# Autodesk Inventor assembly: Shoulder base
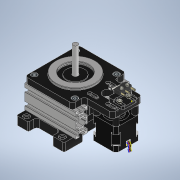
[picture p0: Inventor's stored thumbnail of the model, 180x180]
Saved by Autodesk Inventor 2022 (Build 260153000, 153)
## iProperties
Created: 2022-03-02
Part Number: Shoulder base
Document SubType Name: Assembly
Designer: JK
Author: JK
## Documents named in this file (23)
- C:\Users\JK\Documents\Inventor\ScaraNema\SCARA-3DP\Parts\Shoulder\Shoulder base.iam
- C:\Users\JK\Documents\Inventor\ScaraNema\SCARA-3DP\Parts\Shoulder\Needle roller bearing\5909K79_1 mm Thick Washer for 45 mm Shaft Diameter Needle-Roller Thrust Bearing.ipt
- C:\Users\JK\Documents\Inventor\ScaraNema\SCARA-3DP\Parts\Shoulder\Needle roller bearing\5909K19_Needle-Roller Thrust Bearing.ipt
- C:\Users\JK\Documents\Inventor\ScaraNema\SCARA-3DP\Parts\Common components\GT2 16 Pulley.ipt
- C:\Users\JK\Documents\Inventor\ScaraNema\SCARA-3DP\Parts\Arm\8x80 mm axis.ipt
- C:\Users\JK\Documents\Inventor\ScaraNema\SCARA-3DP\Parts\Common components\GT260T.ipt
- C:\Users\JK\Documents\Inventor\ScaraNema\SCARA-3DP\Parts\Common components\Motor.ipt
- C:\Users\JK\Documents\Inventor\ScaraNema\SCARA-3DP\Parts\Shoulder\Shoulder top base.ipt
- C:\Users\JK\Documents\Inventor\ScaraNema\SCARA-3DP\Parts\Shoulder\shoulder motor separator.ipt
- C:\Users\JK\Documents\Inventor\ScaraNema\SCARA-3DP\Parts\Fasteners\M5 Hex nut.ipt
- C:\Users\JK\Documents\Inventor\ScaraNema\SCARA-3DP\Parts\Shoulder\Arm limit switch support.ipt
- C:\Users\JK\Documents\Inventor\ScaraNema\SCARA-3DP\Parts\Common components\Limit switch.ipt
- C:\Users\JK\Documents\Inventor\ScaraNema\SCARA-3DP\Parts\Fasteners\M3x25 socket solt.ipt
- C:\Users\JK\Documents\Inventor\ScaraNema\SCARA-3DP\Parts\Fasteners\M3 Hex nut.ipt
- C:\Users\JK\Documents\Inventor\ScaraNema\SCARA-3DP\Parts\Fasteners\M5x12 Flat head bolt.ipt
- C:\Users\JK\Documents\Inventor\ScaraNema\SCARA-3DP\Parts\Fasteners\M5x45 Flat head bolt.ipt
- C:\Users\JK\Documents\Inventor\ScaraNema\SCARA-3DP\Parts\Fasteners\M5 T-Nut Drop-in 20x20.ipt
- C:\Users\JK\Documents\Inventor\ScaraNema\SCARA-3DP\Parts\Fasteners\M3x15 socket bolt.ipt
- C:\Users\JK\Documents\Inventor\ScaraNema\SCARA-3DP\Parts\Fasteners\M2 Hex nut.ipt
- C:\Users\JK\Documents\Inventor\ScaraNema\SCARA-3DP\Parts\Fasteners\M2x10 socket bolt.ipt
- C:\Users\JK\Documents\Inventor\ScaraNema\SCARA-3DP\Parts\Common components\688-2RS.ipt
- C:\Users\JK\Documents\Inventor\ScaraNema\SCARA-3DP\Parts\Shoulder\V-Slot 20x40x85.ipt
- C:\Users\JK\Documents\Inventor\ScaraNema\SCARA-3DP\Parts\Shoulder\Shoulder base.ipt
## Components (47 placed, 22 different names)
1. 5909K79_1 mm Thick Washer for 45 mm Shaft Diameter Needle-Roller Thrust Bearing:1 — Tangente:1, Coincidencia:45, Coincidencia:51
2. 5909K19_Needle-Roller Thrust Bearing:1 — Tangente:1, Tangente:2, Coincidencia:45, Coincidencia:46
3. 5909K79_1 mm Thick Washer for 45 mm Shaft Diameter Needle-Roller Thrust Bearing:2 — Tangente:2, Coincidencia:148
4. 8x80 mm axis:1 — Coincidencia:41, Coincidencia:46, Coincidencia:50, Coincidencia:144, Coincidencia:145, Coincidencia:148, Coincidencia:151, Nivelación:47
5. GT260T:1 — Coincidencia:41, Coincidencia:62, Nivelación:17
6. Motor:1 — Ángulo:4, Coincidencia:68, Coincidencia:70, Coincidencia:153
7. GT2 16 Pulley:2 — Nivelación:17, Coincidencia:68, Coincidencia:72
8. Shoulder top base:1 — Coincidencia:50, Coincidencia:51, Ángulo:3, Ángulo:4, Coincidencia:62, Coincidencia:71, Coincidencia:72, Coincidencia:78, Ángulo:7, Nivelación:20, Ángulo:8, Coincidencia:91, Coincidencia:92, Coincidencia:93, Coincidencia:94, Coincidencia:95, Coincidencia:102, Coincidencia:103, Coincidencia:105, Coincidencia:109, Coincidencia:119, Coincidencia:120, Ángulo:14, Coincidencia:121, Coincidencia:122, Coincidencia:123, Coincidencia:146, Coincidencia:149, Nivelación:42, Nivelación:43, Coincidencia:150, Nivelación:45, Nivelación:46
9. Arm limit switch support:1 — Coincidencia:78, Coincidencia:80, Coincidencia:81, Ángulo:6, Ángulo:7, Nivelación:20, Ángulo:8, Coincidencia:124, Ángulo:20, Coincidencia:140, Nivelación:46
10. Limit switch:1 — Coincidencia:80, Coincidencia:81, Ángulo:6, Coincidencia:138, Coincidencia:139, Coincidencia:141, Coincidencia:142, Coincidencia:143
11. M5x12 Flat head bolt:1 — Coincidencia:92, Nivelación:24, Nivelación:25, Coincidencia:95, Coincidencia:111
12. M5x12 Flat head bolt:2 — Coincidencia:93, Nivelación:25, Coincidencia:112
13. M5x12 Flat head bolt:3 — Coincidencia:91, Nivelación:23, Nivelación:24, Coincidencia:110
14. M5x12 Flat head bolt:4 — Coincidencia:94, Nivelación:23, Coincidencia:108
15. M5 T-Nut Drop-in 20x20:2 — Nivelación:28, Nivelación:29, Nivelación:30, Coincidencia:111
16. M5 T-Nut Drop-in 20x20:3 — Nivelación:30, Coincidencia:110
17. M5 T-Nut Drop-in 20x20:4 — Nivelación:29, Coincidencia:112
18. M5 T-Nut Drop-in 20x20:1 — Coincidencia:108, Coincidencia:109, Nivelación:28
19. M3 Hex nut:3 — Coincidencia:119, Nivelación:33, Ángulo:13
20. M3 Hex nut:4 — Coincidencia:120, Nivelación:33, Ángulo:13, Ángulo:14, Coincidencia:121
21. M3x15 socket bolt:1 — Coincidencia:122, Nivelación:34, Coincidencia:124
22. M3x15 socket bolt:2 — Coincidencia:123, Nivelación:34
23. M2 Hex nut:1 — Coincidencia:138, Ángulo:19, Ángulo:20, Nivelación:40, Coincidencia:140
24. M2 Hex nut:2 — Coincidencia:139, Ángulo:19, Nivelación:40
25. M2x10 socket bolt:1 — Coincidencia:141, Nivelación:41, Coincidencia:143
26. M2x10 socket bolt:2 — Coincidencia:142, Nivelación:41
27. 688-2RS:1 — Coincidencia:144, Coincidencia:154
28. 688-2RS:2 — Coincidencia:145, Coincidencia:146
29. V-Slot 20x40x85:1 — Coincidencia:149, Nivelación:42, Nivelación:43, Nivelación:44
30. V-Slot 20x40x85:2 — Coincidencia:150, Nivelación:44, Nivelación:45, Ángulo:21, Coincidencia:152
31. Shoulder base:1 — Coincidencia:151, Ángulo:21, Coincidencia:152, Nivelación:47, Coincidencia:154
32. shoulder motor separator:1 — Coincidencia:70, Coincidencia:71, Coincidencia:104
33. shoulder motor separator:2
34. shoulder motor separator:3
35. shoulder motor separator:4 — Coincidencia:153
36. M5 Hex nut:2
37. M5 Hex nut:3
38. M5 Hex nut:4
39. M5 Hex nut:5
40. M5x45 Flat head bolt:1 — Coincidencia:102, Coincidencia:103
41. M5x45 Flat head bolt:2
42. M5x45 Flat head bolt:3
43. M5x45 Flat head bolt:4
44. M3x25 socket solt:3 — Coincidencia:104, Coincidencia:105
45. M3x25 socket solt:4
46. M3x25 socket solt:5
47. M3x25 socket solt:6
## Component patterns: (4 elements, first: shoulder motor separator:1), (4 elements, first: M5 Hex nut:2), (4 elements, first: M5x45 Flat head bolt:1), (4 elements, first: M3x25 socket solt:3)
## Relationships (79: Mate 49, Flush 18, Angle 10, Tangent 2)
- Tangente:1: 5909K79_1 mm Thick Washer for 45 mm Shaft Diameter Needle-Roller Thrust Bearing:1 ↔ 5909K19_Needle-Roller Thrust Bearing:1
- Tangente:2: 5909K19_Needle-Roller Thrust Bearing:1 ↔ 5909K79_1 mm Thick Washer for 45 mm Shaft Diameter Needle-Roller Thrust Bearing:2
- Coincidencia:41 [Mate]: 8x80 mm axis:1 ↔ GT260T:1
- Coincidencia:45 [Mate]: 5909K79_1 mm Thick Washer for 45 mm Shaft Diameter Needle-Roller Thrust Bearing:1 ↔ 5909K19_Needle-Roller Thrust Bearing:1
- Coincidencia:46 [Mate]: 5909K19_Needle-Roller Thrust Bearing:1 ↔ 8x80 mm axis:1
- Coincidencia:50 [Mate]: 8x80 mm axis:1 ↔ Shoulder top base:1
- Coincidencia:51 [Mate]: 5909K79_1 mm Thick Washer for 45 mm Shaft Diameter Needle-Roller Thrust Bearing:1 ↔ Shoulder top base:1
- Ángulo:3 [Angle] (0 deg): Shoulder top base:1
- Ángulo:4 [Angle] (0 deg): Motor:1 ↔ Shoulder top base:1
- Coincidencia:62 [Mate] (1 mm): GT260T:1 ↔ Shoulder top base:1
- Nivelación:17 [Flush]: GT260T:1 ↔ GT2 16 Pulley:2
- Coincidencia:68 [Mate]: Motor:1 ↔ GT2 16 Pulley:2
- Coincidencia:70 [Mate]: Motor:1 ↔ shoulder motor separator:1
- Coincidencia:71 [Mate]: Shoulder top base:1 ↔ shoulder motor separator:1
- Coincidencia:72 [Mate]: GT2 16 Pulley:2 ↔ Shoulder top base:1
- Coincidencia:78 [Mate]: Shoulder top base:1 ↔ Arm limit switch support:1
- Coincidencia:80 [Mate]: Arm limit switch support:1 ↔ Limit switch:1
- Coincidencia:81 [Mate]: Arm limit switch support:1 ↔ Limit switch:1
- Ángulo:6 [Angle] (0 deg): Arm limit switch support:1 ↔ Limit switch:1
- Ángulo:7 [Angle] (0 deg): Shoulder top base:1 ↔ Arm limit switch support:1
- Nivelación:20 [Flush] (12.5 mm): Shoulder top base:1 ↔ Arm limit switch support:1
- Ángulo:8 [Angle] (0 deg): Shoulder top base:1 ↔ Arm limit switch support:1
- Coincidencia:91 [Mate]: Shoulder top base:1 ↔ M5x12 Flat head bolt:3
- Coincidencia:92 [Mate]: Shoulder top base:1 ↔ M5x12 Flat head bolt:1
- Coincidencia:93 [Mate]: Shoulder top base:1 ↔ M5x12 Flat head bolt:2
- Coincidencia:94 [Mate]: Shoulder top base:1 ↔ M5x12 Flat head bolt:4
- Nivelación:23 [Flush]: M5x12 Flat head bolt:3 ↔ M5x12 Flat head bolt:4
- Nivelación:24 [Flush]: M5x12 Flat head bolt:1 ↔ M5x12 Flat head bolt:3
- Nivelación:25 [Flush]: M5x12 Flat head bolt:1 ↔ M5x12 Flat head bolt:2
- Coincidencia:95 [Mate]: Shoulder top base:1 ↔ M5x12 Flat head bolt:1
- Coincidencia:102 [Mate]: Shoulder top base:1 ↔ M5x45 Flat head bolt:1
- Coincidencia:103 [Mate]: Shoulder top base:1 ↔ M5x45 Flat head bolt:1
- Coincidencia:104 [Mate]: shoulder motor separator:1 ↔ M3x25 socket solt:3
- Coincidencia:105 [Mate]: Shoulder top base:1 ↔ M3x25 socket solt:3
- Coincidencia:108 [Mate]: M5x12 Flat head bolt:4 ↔ M5 T-Nut Drop-in 20x20:1
- Coincidencia:109 [Mate] (0.6 mm): Shoulder top base:1 ↔ M5 T-Nut Drop-in 20x20:1
- Nivelación:28 [Flush]: M5 T-Nut Drop-in 20x20:2 ↔ M5 T-Nut Drop-in 20x20:1
- Nivelación:29 [Flush]: M5 T-Nut Drop-in 20x20:2 ↔ M5 T-Nut Drop-in 20x20:4
- Nivelación:30 [Flush]: M5 T-Nut Drop-in 20x20:2 ↔ M5 T-Nut Drop-in 20x20:3
- Coincidencia:110 [Mate]: M5x12 Flat head bolt:3 ↔ M5 T-Nut Drop-in 20x20:3
- Coincidencia:111 [Mate]: M5x12 Flat head bolt:1 ↔ M5 T-Nut Drop-in 20x20:2
- Coincidencia:112 [Mate]: M5x12 Flat head bolt:2 ↔ M5 T-Nut Drop-in 20x20:4
- Coincidencia:119 [Mate]: Shoulder top base:1 ↔ M3 Hex nut:3
- Coincidencia:120 [Mate]: Shoulder top base:1 ↔ M3 Hex nut:4
- Nivelación:33 [Flush]: M3 Hex nut:3 ↔ M3 Hex nut:4
- Ángulo:13 [Angle] (0 deg): M3 Hex nut:3 ↔ M3 Hex nut:4
- Ángulo:14 [Angle] (0 deg): Shoulder top base:1 ↔ M3 Hex nut:4
- Coincidencia:121 [Mate]: Shoulder top base:1 ↔ M3 Hex nut:4
- Coincidencia:122 [Mate]: Shoulder top base:1 ↔ M3x15 socket bolt:1
- Coincidencia:123 [Mate]: Shoulder top base:1 ↔ M3x15 socket bolt:2
- Nivelación:34 [Flush]: M3x15 socket bolt:1 ↔ M3x15 socket bolt:2
- Coincidencia:124 [Mate]: Arm limit switch support:1 ↔ M3x15 socket bolt:1
- Coincidencia:138 [Mate]: Limit switch:1 ↔ M2 Hex nut:1
- Coincidencia:139 [Mate]: Limit switch:1 ↔ M2 Hex nut:2
- Ángulo:19 [Angle] (0 deg): M2 Hex nut:1 ↔ M2 Hex nut:2
- Ángulo:20 [Angle] (0 deg): Arm limit switch support:1 ↔ M2 Hex nut:1
- Nivelación:40 [Flush]: M2 Hex nut:1 ↔ M2 Hex nut:2
- Coincidencia:140 [Mate]: Arm limit switch support:1 ↔ M2 Hex nut:1
- Coincidencia:141 [Mate]: Limit switch:1 ↔ M2x10 socket bolt:1
- Coincidencia:142 [Mate]: Limit switch:1 ↔ M2x10 socket bolt:2
- Nivelación:41 [Flush]: M2x10 socket bolt:1 ↔ M2x10 socket bolt:2
- Coincidencia:143 [Mate]: Limit switch:1 ↔ M2x10 socket bolt:1
- Coincidencia:144 [Mate]: 8x80 mm axis:1 ↔ 688-2RS:1
- Coincidencia:145 [Mate]: 8x80 mm axis:1 ↔ 688-2RS:2
- Coincidencia:146 [Mate]: Shoulder top base:1 ↔ 688-2RS:2
- Coincidencia:148 [Mate]: 5909K79_1 mm Thick Washer for 45 mm Shaft Diameter Needle-Roller Thrust Bearing:2 ↔ 8x80 mm axis:1
- Coincidencia:149 [Mate]: Shoulder top base:1 ↔ V-Slot 20x40x85:1
- Nivelación:42 [Flush]: Shoulder top base:1 ↔ V-Slot 20x40x85:1
- Nivelación:43 [Flush]: Shoulder top base:1 ↔ V-Slot 20x40x85:1
- Coincidencia:150 [Mate]: Shoulder top base:1 ↔ V-Slot 20x40x85:2
- Nivelación:44 [Flush]: V-Slot 20x40x85:1 ↔ V-Slot 20x40x85:2
- Nivelación:45 [Flush]: Shoulder top base:1 ↔ V-Slot 20x40x85:2
- Coincidencia:151 [Mate]: 8x80 mm axis:1 ↔ Shoulder base:1
- Ángulo:21 [Angle] (0 deg): V-Slot 20x40x85:2 ↔ Shoulder base:1
- Coincidencia:152 [Mate]: V-Slot 20x40x85:2 ↔ Shoulder base:1
- Nivelación:46 [Flush] (-5 mm): Shoulder top base:1 ↔ Arm limit switch support:1
- Coincidencia:153 [Mate]: Motor:1 ↔ shoulder motor separator:4
- Nivelación:47 [Flush] (28 mm): 8x80 mm axis:1 ↔ Shoulder base:1
- Coincidencia:154 [Mate]: 688-2RS:1 ↔ Shoulder base:1
